# Autodesk Inventor assembly: Extruder Midbody Assembly
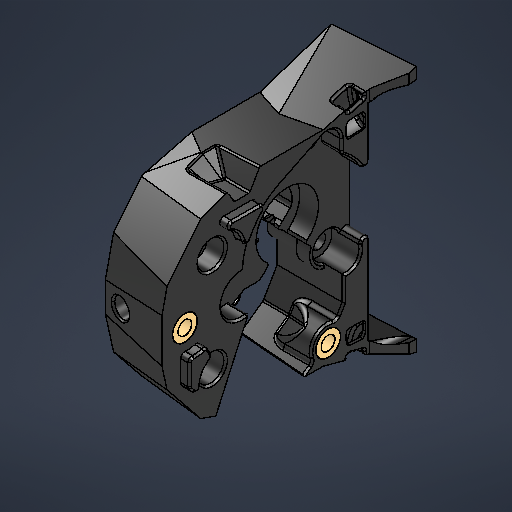
[picture p0: Inventor's stored thumbnail of the model, 512x512]
Saved by Autodesk Inventor 2026 (Build 300175050, 175E)
## iProperties
Created: 2025-05-11
Part Number: Extruder Midbody Assembly
Document SubType Name: Assembly
Designer: Joshua Eah
Author: Joshua Eah
## Documents named in this file (4)
- C:\Users\Joshua Eah\Documents\GitHub\Voron-0\CAD\Master Assembly\Toolhead\Subassemblies\Extruder Midbody Assembly.iam
- C:\Users\Joshua Eah\Documents\GitHub\Voron-0\CAD\Master Assembly\Hardware\M2x6 FHCS.ipt
- C:\Users\Joshua Eah\Documents\GitHub\Voron-0\CAD\Master Assembly\Toolhead\Parts\Extruder Midbody.ipt
- C:\Users\Joshua Eah\Documents\GitHub\Voron-0\CAD\Master Assembly\Hardware\M3 Threaded Insert.ipt
## Components (7 placed, 3 different names)
1. M2x6 FHCS:1 — Mate:1
2. Extruder Midbody:1 — Mate:1, Insert:1, Insert:2, Insert:3, Insert:4, Insert:5
3. M3 Threaded Insert:1 — Insert:4
4. M3 Threaded Insert:2 — Insert:5
5. M3 Threaded Insert:3 — Insert:3
6. M3 Threaded Insert:4 — Insert:2
7. M3 Threaded Insert:5 — Insert:1
## Relationships (6: Insert 5, Mate 1)
- Mate:1: M2x6 FHCS:1 ↔ Extruder Midbody:1
- Insert:1: Extruder Midbody:1 ↔ M3 Threaded Insert:5
- Insert:2: Extruder Midbody:1 ↔ M3 Threaded Insert:4
- Insert:3: Extruder Midbody:1 ↔ M3 Threaded Insert:3
- Insert:4: Extruder Midbody:1 ↔ M3 Threaded Insert:1
- Insert:5: Extruder Midbody:1 ↔ M3 Threaded Insert:2
